# Autodesk Inventor assembly: Cup_Dispenser_Dynamic
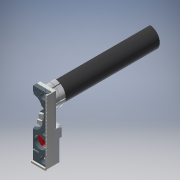
[picture p0: Inventor's stored thumbnail of the model, 180x180]
Saved by Autodesk Inventor 2016 (Build 200138000, 138)
## iProperties
Electromechanical_EMX_Project: C:\Users\3DPrinterUser\Documents\GitHub\BarBot\Conception\Mechanical\Cup_Dispenser_Dynamic\cabling.emx
Electromechanical_Physical_Snapshot: C:\Users\3DPrinterUser\Documents\GitHub\BarBot\Conception\Mechanical\Cup_Dispenser_Dynamic\cabling_Physical.snapshot
Electromechanical_Logical_Snapshot: C:\Users\3DPrinterUser\Documents\GitHub\BarBot\Conception\Mechanical\Cup_Dispenser_Dynamic\cabling_Logical.snapshot
Electromechanical_Vault_Folder: EMX\{F2857C4D-FD79-4659-B156-E1495D173BB8}
_MechatronicsProject: <Project Version="1.0"><Path>C:\Users\3DPrinterUser\Documents\GitHub\BarBot\Conception\Mechanical\Cup_Dispenser_Dynamic\cabling.emx</Path><Guid>{F2857C4D-FD79-4659-B156-E1495D173BB8}</Guid><IPJFileName>C:\Users\Public\Documents\Autodesk\Inventor 2016\Default.ipj</IPJFileName><IPJWorkFolder></IPJWorkFolder><AssemblyFileName>C:\Users\3DPrinterUser\Documents\GitHub\BarBot\Conception\Mechanical\Cup_Dispenser_Dynamic\Cup_Dispenser_Dynamic.iam</AssemblyFileName><AssemblyFileGUID>{0E46BEC1-E96B-4DE1-BEFF-2BDC7A836DF8}</AssemblyFileGUID></Project>
_MTAssemblyInfoProperty: <MechatronicsAssembly Version="1.0" ID="{0E46BEC1-E96B-4DE1-BEFF-2BDC7A836DF8}"><MechatronicsComponents/><MechatronicsComponentDefs/><MechatronicsHarnessAssemblies/><MechatronicsConnectionDefs/><MechatronicsConnections/><MechatronicsCableDefs/><MechatronicsCables/><MechatronicsSubAssemblies/><ComponentLinks/><MechatronicsAssemblyRevision FileRevision="35"><Occurrences><Occurrence FileName="C:\Users\3DPrinterUser\Documents\GitHub\BarBot\Conception\Mechanical\Cup_Dispenser\Cup_Dispenser_Pipe.ipt" Name="Cup_Dispenser_Pipe:1" FileRevision="{91B701CC-AD9C-7788-BF8F-6A49EB822AEB}"/><Occurrence FileName="C:\Users\3DPrinterUser\Documents\GitHub\BarBot\Conception\Mechanical\Cup_Dispenser_Dynamic\Board.ipt" Name="Board:1" FileRevision="{692E8835-ECF1-96CA-79BB-E2E8D7CD61F8}"/><Occurrence FileName="C:\Users\3DPrinterUser\Documents\GitHub\BarBot\Conception\Mechanical\Cup_Dispenser_Dynamic\Cup_Dispenser_Fixture.ipt" Name="Cup_Dispenser_Fixture:1" FileRevision="{AB585B0A-CC2D-16C7-F03A-E315701848A4}"/><Occurrence FileName="C:\Users\3DPrinterUser\Documents\GitHub\BarBot\Conception\Mechanical\Cup_Dispenser_Dynamic\Cup_Dispenser_Hull.ipt" Name="Cup_Dispenser_Hull:1" FileRevision="{A9F2E11E-482E-074A-7AF9-082168FED3DF}"/><Occurrence FileName="C:\Users\3DPrinterUser\Documents\GitHub\BarBot\Conception\Mechanical\Cup_Dispenser_Dynamic\Cup_Dispenser_Slider.ipt" Name="Cup_Dispenser_Slider:1" FileRevision="{A70251B8-3810-9E15-D18F-2092E07F01C6}"/><Occurrence FileName="C:\Users\3DPrinterUser\Documents\GitHub\BarBot\Conception\Mechanical\Cup_Dispenser_Dynamic\Cup_Dispenser_Stepper_Montage.ipt" Name="Cup_Dispenser_Stepper_Montage:1" FileRevision="{E6DF2F95-AF89-29CA-14F1-C13E5F5175B5}"/><Occurrence FileName="C:\Users\3DPrinterUser\Documents\GitHub\BarBot\Conception\Mechanical\Cup_Dispenser_Dynamic\Cup_Dispenser_Transmission.ipt" Name="Cup_Dispenser_Transmission:1" FileRevision=""/><Occurrence FileName="C:\Users\3DPrinterUser\Documents\GitHub\BarBot\Conception\Mechanical\Cup_Dispenser_Dynamic\M1173041- NEMA 17.ipt" Name="M1173041- NEMA 17:1" FileRevision="{D043204F-FB44-6E63-5DB6-AE93EB722DB9}"/></Occurrences></MechatronicsAssemblyRevision></MechatronicsAssembly>
Created: 2015-07-09
Part Number: Cup_Dispenser_Dynamic
Document SubType Name: Assembly
Designer: marku
Author: marku
## Documents named in this file (9)
- C:\Users\3DPrinterUser\Documents\GitHub\BarBot\Conception\Mechanical\Cup_Dispenser_Dynamic\Cup_Dispenser_Dynamic.iam
- C:\Users\3DPrinterUser\Documents\GitHub\BarBot\Conception\Mechanical\Cup_Dispenser_Dynamic\Cup_Dispenser_Hull.ipt
- C:\Users\3DPrinterUser\Documents\GitHub\BarBot\Conception\Mechanical\Cup_Dispenser_Dynamic\Cup_Dispenser_Fixture.ipt
- C:\Users\3DPrinterUser\Documents\GitHub\BarBot\Conception\Mechanical\Cup_Dispenser_Dynamic\Cup_Dispenser_Stepper_Montage.ipt
- C:\Users\3DPrinterUser\Documents\GitHub\BarBot\Conception\Mechanical\Cup_Dispenser_Dynamic\M1173041- NEMA 17.ipt
- C:\Users\3DPrinterUser\Documents\GitHub\BarBot\Conception\Mechanical\Cup_Dispenser_Dynamic\Cup_Dispenser_Slider.ipt
- C:\Users\3DPrinterUser\Documents\GitHub\BarBot\Conception\Mechanical\Cup_Dispenser_Dynamic\Cup_Dispenser_Transmission.ipt
- C:\Users\3DPrinterUser\Documents\GitHub\BarBot\Conception\Mechanical\Cup_Dispenser\Cup_Dispenser_Pipe.ipt
- C:\Users\3DPrinterUser\Documents\GitHub\BarBot\Conception\Mechanical\Cup_Dispenser_Dynamic\Board.ipt
## Components (8 placed, 8 different names)
1. Cup_Dispenser_Hull:1 — Flush:1, Flush:2, Flush:3
2. Cup_Dispenser_Fixture:1 — Flush:1, Rotational:1
3. Cup_Dispenser_Stepper_Montage:1 — Flush:2, Rigid:1, Flush:6, Flush:7
4. M1173041- NEMA 17:1 — Rigid:1, Flush:5
5. Cup_Dispenser_Slider:1 — Flush:3, Flush:4
6. Cup_Dispenser_Transmission:1 — Flush:4, Flush:5
7. Cup_Dispenser_Pipe:1 — Rotational:1
8. Board:1 — Flush:6, Flush:7
## Relationships (9: Flush 7, WeldJoint 1, RevoluteJoint 1)
- Flush:1: Cup_Dispenser_Hull:1 ↔ Cup_Dispenser_Fixture:1
- Flush:2: Cup_Dispenser_Hull:1 ↔ Cup_Dispenser_Stepper_Montage:1
- Rigid:1 [WeldJoint]: Cup_Dispenser_Stepper_Montage:1 ↔ M1173041- NEMA 17:1
- Flush:3: Cup_Dispenser_Hull:1 ↔ Cup_Dispenser_Slider:1
- Flush:4: Cup_Dispenser_Slider:1 ↔ Cup_Dispenser_Transmission:1
- Flush:5: M1173041- NEMA 17:1 ↔ Cup_Dispenser_Transmission:1
- Rotational:1 [RevoluteJoint]: Cup_Dispenser_Fixture:1 ↔ Cup_Dispenser_Pipe:1
- Flush:6: Cup_Dispenser_Stepper_Montage:1 ↔ Board:1
- Flush:7 (6 mm): Cup_Dispenser_Stepper_Montage:1 ↔ Board:1
